# Autodesk Inventor assembly: Transmission par courroie trapézoïdale
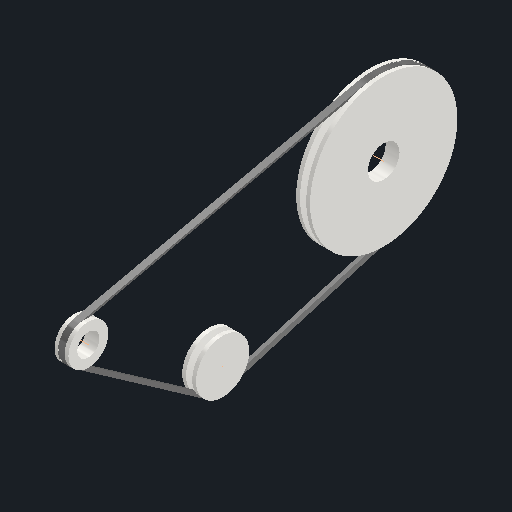
[picture p0: Inventor's stored thumbnail of the model, 512x512]
Saved by Autodesk Inventor 2026.2 (Build 302298010, 298A)
## iProperties
ClientObjectVersion: 1
Created: 2026-03-31
Part Number: Transmission par courroie trapézoïdale
Document SubType Name: Assembly
Designer: romai
Author: romai
## Documents named in this file (5)
- D:\Downloads\LogicielMaster\Inventor\Enssemble\BancEcoShell\BancEcoShell\Design Accelerator\Transmission par courroie trapézoïdale2.iam
- D:\Downloads\LogicielMaster\Inventor\Enssemble\BancEcoShell\BancEcoShell\Design Accelerator\Courroie trapézoïdale2.ipt
- D:\Downloads\LogicielMaster\Inventor\Enssemble\BancEcoShell\BancEcoShell\Design Accelerator\Poulie à gorge12.ipt
- D:\Downloads\LogicielMaster\Inventor\Enssemble\BancEcoShell\BancEcoShell\Design Accelerator\Poulie à gorge22.ipt
- D:\Downloads\LogicielMaster\Inventor\Enssemble\BancEcoShell\BancEcoShell\Design Accelerator\Poulie à gorge32.ipt
## Components (4 placed, 4 different names)
1. Poulie à gorge1:1 — Affleurement:1, Placage:1, Rotation:1, Rotation:2
2. Poulie à gorge2:1 — Affleurement:2, Placage:2, Rotation:1
3. Poulie à gorge3:1 — Affleurement:3, Placage:3, Rotation:2
4. Courroie trapézoïdale:1 — Affleurement:1, Placage:1, Affleurement:2, Placage:2, Affleurement:3, Placage:3
## Component patterns: (1 elements, first: Courroie trapézoïdale:1)
## Relationships (8: Flush 3, Mate 3, RelateRotation 2)
- Affleurement:1 [Flush]: Poulie à gorge1:1 ↔ Courroie trapézoïdale:1
- Placage:1 [Mate]: Poulie à gorge1:1 ↔ Courroie trapézoïdale:1
- Affleurement:2 [Flush]: Poulie à gorge2:1 ↔ Courroie trapézoïdale:1
- Placage:2 [Mate]: Poulie à gorge2:1 ↔ Courroie trapézoïdale:1
- Rotation:1 [RelateRotation] (0.2576 ul): Poulie à gorge1:1 ↔ Poulie à gorge2:1
- Affleurement:3 [Flush]: Poulie à gorge3:1 ↔ Courroie trapézoïdale:1
- Placage:3 [Mate]: Poulie à gorge3:1 ↔ Courroie trapézoïdale:1
- Rotation:2 [RelateRotation] (0.3493 ul): Poulie à gorge1:1 ↔ Poulie à gorge3:1
